# Autodesk Inventor assembly: Assembly1 dolorimetro final
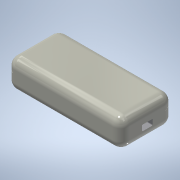
[picture p0: Inventor's stored thumbnail of the model, 180x180]
Saved by Autodesk Inventor 2022 (Build 260153000, 153)
## iProperties
Created: 2022-11-14
Part Number: Assembly1 dolorimetro final
Document SubType Name: Assembly
Designer: ASUS
Author: ASUS
## Documents named in this file (3)
- C:\CICLO IV\FUNDAMENTOS DE BIODISEÑO\BIODEÑO\Assembly1 dolorimetro final.iam
- C:\CICLO IV\FUNDAMENTOS DE BIODISEÑO\BIODEÑO\CARCASA NUEVA (2).ipt
- C:\CICLO IV\FUNDAMENTOS DE BIODISEÑO\BIODEÑO\CARCASA NUEVA ARRIBA 1411.ipt
## Components (2 placed, 2 different names)
1. CARCASA NUEVA (2):1 — Flush:1, Mate:1, Mate:2
2. CARCASA NUEVA ARRIBA 1411:1 — Flush:1, Mate:1, Mate:2
## Relationships (3: Mate 2, Flush 1)
- Flush:1: CARCASA NUEVA (2):1 ↔ CARCASA NUEVA ARRIBA 1411:1
- Mate:1: CARCASA NUEVA (2):1 ↔ CARCASA NUEVA ARRIBA 1411:1
- Mate:2: CARCASA NUEVA (2):1 ↔ CARCASA NUEVA ARRIBA 1411:1
